# Autodesk Inventor assembly: wheel_ass_2
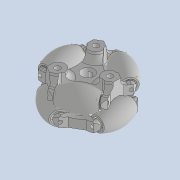
[picture p0: Inventor's stored thumbnail of the model, 180x180]
Saved by Autodesk Inventor 2020 (Build 240168000, 168)
## iProperties
Created: 2022-01-11
Part Number: wheel_ass_2
Document SubType Name: Assembly
Designer: Shuang Peng
Author: Shuang Peng
## Documents named in this file (5)
- D:\projects-3\soft module robot\hardware\diff module 3\wheel_ass_2.iam
- D:\projects-3\soft module robot\hardware\diff module 3\wheel_2.ipt
- D:\projects-3\soft module robot\hardware\diff module 3\roller_2.ipt
- D:\projects-3\soft module robot\hardware\diff module 3\beraing_1_3_1.ipt
- D:\projects-3\soft module robot\hardware\diff module 3\wheel_3.ipt
## Components (14 placed, 4 different names)
1. wheel_2:1 — Insert:7, Insert:8, Insert:9, Insert:10, Insert:11
2. roller_2:1 — Insert:1, Insert:2
3. beraing_1_3_1:1 — Insert:2
4. beraing_1_3_1:2 — Insert:1, Insert:9
5. roller_2:2
6. beraing_1_3_1:3
7. beraing_1_3_1:4 — Insert:7
8. roller_2:3
9. beraing_1_3_1:5
10. beraing_1_3_1:6 — Insert:8
11. wheel_3:1 — Insert:10, Insert:11, Insert:12, Insert:13, Insert:14
12. roller_2:4 — Insert:14
13. roller_2:5 — Insert:13
14. roller_2:6 — Insert:12
## Relationships (14: Insert 14)
- Insert:1 (-0.1 mm): roller_2:1 ↔ beraing_1_3_1:2
- Insert:2: roller_2:1 ↔ beraing_1_3_1:1
- [Insert] (-0.1 mm): roller_2:2 ↔ beraing_1_3_1:4
- [Insert]: roller_2:2 ↔ beraing_1_3_1:3
- [Insert] (-0.1 mm): roller_2:3 ↔ beraing_1_3_1:6
- [Insert]: roller_2:3 ↔ beraing_1_3_1:5
- Insert:7: wheel_2:1 ↔ beraing_1_3_1:4
- Insert:8: wheel_2:1 ↔ beraing_1_3_1:6
- Insert:9: wheel_2:1 ↔ beraing_1_3_1:2
- Insert:10: wheel_2:1 ↔ wheel_3:1
- Insert:11: wheel_2:1 ↔ wheel_3:1
- Insert:12 (0.1 mm): wheel_3:1 ↔ roller_2:6
- Insert:13 (0.1 mm): wheel_3:1 ↔ roller_2:5
- Insert:14 (0.1 mm): wheel_3:1 ↔ roller_2:4
## Named parameters: d2_d0 = -0.1 mm, d3_d1 = 0 mm, d4_d0 = -0.1 mm, d5_d1 = 0 mm
